# Autodesk Inventor assembly: NewChassis
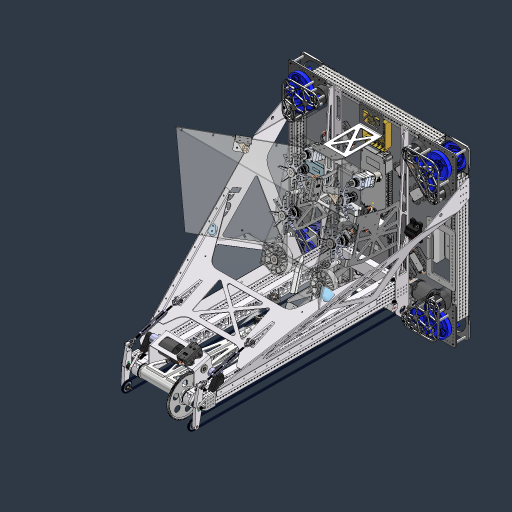
[picture p0: Inventor's stored thumbnail of the model, 512x512]
Saved by Autodesk Inventor 2024.3 (Build 283343000, 343)
## iProperties
ILogicPurgeVersion: 0.0.0.0
OnSaveVersion: 3.5.0.0
OnSaveAssembly: COREAutomationManager
Created: 2025-01-13
Part Number: NewChassis
Document SubType Name: Assembly
Designer: Marcus Tannini
Mfg Approved By: John.Thibert
Mass: 34331.5 g
Surface Area: 95241.2 cm^2
Volume: 13545.5 cm^3
Density: 2.53453 g/cm^3
ModelCat: Uncategorized
CN_MASS: 68.7
Author: Marcus Tannini
## Documents named in this file (42)
- D:\Inventor Projects\Poseidon V2\#Poseidon 2025.iam
- D:\Inventor Projects\Poseidon V2\ASSY,MK4i,Swerve_Module_INV.iam
- D:\Inventor Projects\Poseidon V2\MAXTube-2x1-Holes.ipt
- D:\Inventor Projects\Poseidon V2\BellyPanTop.ipt
- D:\Inventor Projects\Poseidon V2\BellyPanBot.ipt
- D:\Inventor Projects\Poseidon V2\BATTERY,12V.ipt
- D:\Inventor Projects\Poseidon V2\CONTROLS,MAIN_BREAKER.ipt
- D:\Inventor Projects\Poseidon V2\CONTROLS,MOTOR,NEO,550.ipt
- D:\Inventor Projects\Poseidon V2\CONTROLS,PDH.ipt
- D:\Inventor Projects\Poseidon V2\CONTROLS,PH.ipt
- D:\Inventor Projects\Poseidon V2\CONTROLS,ROBO_RIO.ipt
- D:\Inventor Projects\Poseidon V2\CONTROLS,SPARK_MAX.ipt
- D:\Inventor Projects\Poseidon V2\CONTROLS,VRM.ipt
- D:\Inventor Projects\Poseidon V2\COVER,SPARKMAX.ipt
- D:\Inventor Projects\Poseidon V2\ModifiedCase(IncludesPatterning).iam
- D:\Inventor Projects\Poseidon V2\PLATE,MOUNT,BATTERY,TOP.ipt
- D:\Inventor Projects\Poseidon V2\PLATE,MOUNT,BATTERY,BOT.ipt
- D:\Inventor Projects\Poseidon V2\MOUNT,STRAP,BATTERY.ipt
- D:\Inventor Projects\Poseidon V2\SPACER,SPROCKET,IDLER,ELEVATOR.ipt
- D:\Inventor Projects\Poseidon V2\PLATE,SIDE,BRACE,RIGHT,ELEVATOR.ipt
- D:\Inventor Projects\Poseidon V2\PLATE,SIDE,BRACE,LEFT,ELEVATOR.ipt
- D:\Inventor Projects\Poseidon V2\PLATE,TURNBUCKLE,TENSIONER,CHAIN.ipt
- D:\Inventor Projects\Poseidon V2\PLATE,BRACE,HORISONTAL,TOP,ELEVATOR.ipt
- D:\Inventor Projects\Poseidon V2\TURNBUCKLE,0.25IN_CLEVIS.iam
- D:\Inventor Projects\Poseidon V2\STAGE1,ELEVATOR.iam
- D:\Inventor Projects\Poseidon V2\ASSY,MAIN,ELEVATOR.iam
- D:\Inventor Projects\Poseidon V2\ANGLE,MOUNT,ELEVATOR.ipt
- D:\Inventor Projects\Poseidon V2\ANGLE,MOUNT,ELEVATOR,MIRR.ipt
- D:\Inventor Projects\Poseidon V2\FABRIC,BUMPERS.ipt
- D:\Inventor Projects\Poseidon V2\9293K119_Constant-Force Spring.ipt
- D:\Inventor Projects\Poseidon V2\MOUNT,SPRING,ELEVATOR.ipt
- D:\Inventor Projects\Poseidon V2\MOUNT,SPRING,ELEVATOR,MIRR.ipt
- D:\Inventor Projects\Poseidon V2\SPACER,HEX,0.125IN.ipt
- D:\Inventor Projects\Poseidon V2\ARM.iam
- D:\Inventor Projects\Poseidon V2\DRIVETRAIN,ELEVATOR.iam
- D:\Inventor Projects\Poseidon V2\hopper_assy.iam
- D:\Inventor Projects\Poseidon V2\feeder_front_support.ipt
- D:\Inventor Projects\Poseidon V2\coral_end_stop.ipt
- D:\Inventor Projects\Poseidon V2\coral_end_stop_MIR.ipt
- D:\Inventor Projects\Poseidon V2\hopper_backboard.ipt
- D:\Inventor Projects\Poseidon V2\Part Studio 1 - Support 1.ipt
- D:\Inventor Projects\Poseidon V2\Part Studio 1 - Support 2.ipt
## Components (67 placed, 43 different names)
1. FABRIC,BUMPERS.ipt:1 — Flush:323, Mate:335, Mate:336
2. hopper_assy:1 [sub-assembly] — Mate:656, Mate:657, Mate:658, Mate:671, Mate:672, Mate:673, Mate:674, Mate:675, Mate:676
3. feeder_front_support:1 — Mate:659, Mate:660, Mate:661, Mate:662, Mate:663, Mate:664, Mate:665, Mate:666, Mate:667
4. coral_end_stop:1 — Mate:665, Mate:666, Mate:667
5. coral_end_stop_MIR:1 — Mate:662, Mate:663, Mate:664
6. hopper_backboard:1 — Mate:668, Mate:669, Mate:670
7. Part Studio 1 - Support 1:1 — Mate:674, Mate:675, Mate:676
8. Part Studio 1 - Support 2:1 — Mate:671, Mate:672, Mate:673
9. ARM:1 [sub-assembly] — GEARS,ARM, Angle:1
10. COVER,SPARKMAX:9
11. CONTROLS,SPARK_MAX:9 — Mate:655
12. BellyPanBot.ipt:1 — Mate:66, Mate:353, Mate:354
13. BellyPanTop.ipt:1 — Mate:62, Mate:63, Mate:65, Mate:70, Mate:71, Mate:82, Mate:84, Insert:7, Insert:8, Insert:9, Insert:10, Insert:11, Insert:12, Insert:13, Insert:14, Insert:15, Insert:16, Insert:17, Insert:18, Insert:19, Insert:20, Insert:21, Insert:22, Mate:111, Mate:113, Mate:114, Mate:116, Mate:117, Mate:118, Mate:119, Mate:121, Mate:122, Mate:123, Mate:124, Mate:125, Mate:126, Mate:127, Mate:130, Insert:23, Insert:24, Mate:308, Mate:320, Mate:349, Mate:350, Mate:659, Mate:660, Mate:661
14. MAXTube-2x1-Holes.ipt:1 — Mate:1, Mate:2, Mate:3, Mate:4, Mate:5, Mate:15, Mate:115, Mate:272
15. MAXTube-2x1-Holes.ipt:2 — Mate:6, Mate:7, Mate:8, Mate:9, Mate:10, Mate:11, Mate:62, Mate:309, Mate:310
16. MAXTube-2x1-Holes.ipt:3 — Mate:19, Mate:20, Mate:21, Mate:66, Mate:114, Mate:312, Mate:313, Mate:336
17. MAXTube-2x1-Holes.ipt:4 — Mate:12, Mate:13, Mate:14, Mate:16, Mate:17, Mate:18, Mate:29, Mate:63, Mate:271, Mate:353, Mate:354
18. MOUNT,STRAP,BATTERY.ipt:1 — Mate:357, Mate:358, Mate:359
19. PLATE,MOUNT,BATTERY,BOT.ipt:1 — Mate:320, Mate:321, Mate:351, Mate:352
20. PLATE,MOUNT,BATTERY,TOP.ipt:1 — Mate:127, Mate:349, Mate:350, Mate:351, Mate:352, Mate:356, Mate:357, Mate:358, Mate:359
21. BATTERY,12V.ipt:1 — Mate:321, Mate:356
22. CONTROLS,MAIN_BREAKER.ipt:1 — Mate:82, Mate:111, Mate:116
23. CONTROLS,MOTOR,NEO,550.ipt:1
24. CONTROLS,PDH.ipt:1 — Mate:113, Mate:117, Mate:118, Mate:119
25. CONTROLS,PH.ipt:1 — Insert:23, Insert:24
26. CONTROLS,ROBO_RIO.ipt:1 — Mate:124, Mate:125, Mate:126
27. CONTROLS,SPARK_MAX.ipt:1 — Mate:84, Mate:85, Mate:86, Mate:87
28. CONTROLS,VRM.ipt:1 — Mate:121, Mate:122, Mate:123
29. ModifiedCase(IncludesPatterning).iam:1 [sub-assembly] — Mate:130
30. ASSY,MAIN,ELEVATOR.iam:1 [sub-assembly] — Mate:161, Mate:162, Flush:19, Mate:297, STAGE1 UPPER LIMIT, STAGE1 MAX, Mate:311, Mate:314, Mate:315, Mate:363, Mate:362, Mate:366, Mate:367, Mate:368, Mate:369
31. DRIVETRAIN,ELEVATOR:1 [sub-assembly]
32. STAGE1,ELEVATOR.iam:1 [sub-assembly] — Flush:19, Mate:297, STAGE1 LOWER LIMIT, STAGE1 UPPER LIMIT, STAGE1 MIN, STAGE1 MAX, GEARS,ARM, Angle:1, Mate:655
33. TURNBUCKLE,0.25IN_CLEVIS.iam:1 [sub-assembly]
34. TURNBUCKLE,0.25IN_CLEVIS.iam:2 [sub-assembly] — Mate:625
35. 9293K119_Constant-Force Spring:1 — Mate:364, Mate:365
36. 9293K119_Constant-Force Spring:2 — Mate:370, Mate:371
37. ANGLE,MOUNT,ELEVATOR,MIRR.ipt:1 — Mate:308, Mate:309, Mate:310, Mate:311, Mate:312, Mate:313, Mate:314, Mate:315, Mate:656, Mate:657, Mate:658
38. ANGLE,MOUNT,ELEVATOR.ipt:1 — Mate:65, Mate:70, Mate:71, Mate:161, Mate:162, STAGE1 LOWER LIMIT, STAGE1 MIN
39. MOUNT,SPRING,ELEVATOR,MIRR:1 — Mate:367, Mate:368, Mate:369, Mate:370, Mate:371
40. MOUNT,SPRING,ELEVATOR:1 — Mate:363, Mate:362, Mate:364, Mate:365, Mate:366
41. PLATE,BRACE,HORISONTAL,TOP,ELEVATOR.ipt:1 — Mate:285, Mate:286, Mate:289, Mate:290, Mate:291, Mate:295, Mate:296, Mate:668, Mate:669, Mate:670
42. PLATE,SIDE,BRACE,LEFT,ELEVATOR.ipt:1 — Mate:271, Mate:289, Mate:290, Mate:291, Mate:335
43. PLATE,SIDE,BRACE,RIGHT,ELEVATOR.ipt:1 — Mate:272
44. PLATE,TURNBUCKLE,TENSIONER,CHAIN.ipt:1 — Mate:285, Mate:296
45. PLATE,TURNBUCKLE,TENSIONER,CHAIN.ipt:2 — Mate:286, Mate:295, Mate:625
46. SPACER,HEX,0.125IN:1
47. SPACER,SPROCKET,IDLER,ELEVATOR.ipt:1
48. SPACER,SPROCKET,IDLER,ELEVATOR.ipt:2
49. ASSY,MK4i,Swerve_Module_INV.iam:1 [sub-assembly] — Mate:1, Mate:2, Mate:15
50. ASSY,MK4i,Swerve_Module_INV.iam:2 [sub-assembly] — Mate:3, Mate:4, Mate:5, Mate:6, Mate:7, Mate:8
51. ASSY,MK4i,Swerve_Module_INV.iam:3 [sub-assembly] — Mate:9, Mate:10, Mate:11, Mate:12, Mate:13, Mate:14
52. ASSY,MK4i,Swerve_Module_INV.iam:4 [sub-assembly] — Mate:16, Mate:17, Mate:18, Mate:19, Mate:20, Mate:21, Mate:67
53. CONTROLS,SPARK_MAX.ipt:2
54. CONTROLS,SPARK_MAX.ipt:3
55. CONTROLS,SPARK_MAX.ipt:4
56. CONTROLS,SPARK_MAX.ipt:5
57. CONTROLS,SPARK_MAX.ipt:6
58. CONTROLS,SPARK_MAX.ipt:7
59. CONTROLS,SPARK_MAX.ipt:8
60. COVER,SPARKMAX.ipt:1 — Mate:85, Mate:86, Mate:87, Insert:7, Insert:8
61. COVER,SPARKMAX.ipt:2 — Insert:9, Insert:10
62. COVER,SPARKMAX.ipt:3 — Insert:11, Insert:12
63. COVER,SPARKMAX.ipt:4 — Insert:13, Insert:14
64. COVER,SPARKMAX.ipt:5 — Insert:17, Insert:18
65. COVER,SPARKMAX.ipt:6 — Insert:15, Insert:16
66. COVER,SPARKMAX.ipt:7 — Insert:21, Insert:22
67. COVER,SPARKMAX.ipt:8 — Insert:19, Insert:20
## Relationships (198: Mate 170, Insert 22, Flush 4, RelateRotation 1, Angle 1)
- Mate:1: MAXTube-2x1-Holes.ipt:1 ↔ ASSY,MK4i,Swerve_Module_INV.iam:1
- Mate:2: MAXTube-2x1-Holes.ipt:1 ↔ ASSY,MK4i,Swerve_Module_INV.iam:1
- Mate:3: MAXTube-2x1-Holes.ipt:1 ↔ ASSY,MK4i,Swerve_Module_INV.iam:2
- Mate:4: MAXTube-2x1-Holes.ipt:1 ↔ ASSY,MK4i,Swerve_Module_INV.iam:2
- Mate:5: MAXTube-2x1-Holes.ipt:1 ↔ ASSY,MK4i,Swerve_Module_INV.iam:2
- Mate:6: MAXTube-2x1-Holes.ipt:2 ↔ ASSY,MK4i,Swerve_Module_INV.iam:2
- Mate:7: MAXTube-2x1-Holes.ipt:2 ↔ ASSY,MK4i,Swerve_Module_INV.iam:2
- Mate:8: MAXTube-2x1-Holes.ipt:2 ↔ ASSY,MK4i,Swerve_Module_INV.iam:2
- Mate:9: MAXTube-2x1-Holes.ipt:2 ↔ ASSY,MK4i,Swerve_Module_INV.iam:3
- Mate:10: MAXTube-2x1-Holes.ipt:2 ↔ ASSY,MK4i,Swerve_Module_INV.iam:3
- Mate:11: MAXTube-2x1-Holes.ipt:2 ↔ ASSY,MK4i,Swerve_Module_INV.iam:3
- Mate:12: MAXTube-2x1-Holes.ipt:4 ↔ ASSY,MK4i,Swerve_Module_INV.iam:3
- Mate:13: MAXTube-2x1-Holes.ipt:4 ↔ ASSY,MK4i,Swerve_Module_INV.iam:3
- Mate:14: MAXTube-2x1-Holes.ipt:4 ↔ ASSY,MK4i,Swerve_Module_INV.iam:3
- Mate:15: MAXTube-2x1-Holes.ipt:1 ↔ ASSY,MK4i,Swerve_Module_INV.iam:1
- Mate:16: MAXTube-2x1-Holes.ipt:4 ↔ ASSY,MK4i,Swerve_Module_INV.iam:4
- Mate:17: MAXTube-2x1-Holes.ipt:4 ↔ ASSY,MK4i,Swerve_Module_INV.iam:4
- Mate:18: MAXTube-2x1-Holes.ipt:4 ↔ ASSY,MK4i,Swerve_Module_INV.iam:4
- Mate:19: MAXTube-2x1-Holes.ipt:3 ↔ ASSY,MK4i,Swerve_Module_INV.iam:4
- Mate:20: MAXTube-2x1-Holes.ipt:3 ↔ ASSY,MK4i,Swerve_Module_INV.iam:4
- Mate:21: MAXTube-2x1-Holes.ipt:3 ↔ ASSY,MK4i,Swerve_Module_INV.iam:4
- Mate:29 (-6.35 mm): MAXTube-2x1-Holes.ipt:4
- Mate:62: BellyPanTop.ipt:1 ↔ MAXTube-2x1-Holes.ipt:2
- Mate:63: BellyPanTop.ipt:1 ↔ MAXTube-2x1-Holes.ipt:4
- Mate:65: BellyPanTop.ipt:1 ↔ ANGLE,MOUNT,ELEVATOR.ipt:1
- Mate:66: BellyPanBot.ipt:1 ↔ MAXTube-2x1-Holes.ipt:3
- Mate:67 (35.56 mm): ASSY,MK4i,Swerve_Module_INV.iam:4
- Mate:70: BellyPanTop.ipt:1 ↔ ANGLE,MOUNT,ELEVATOR.ipt:1
- Mate:71: BellyPanTop.ipt:1 ↔ ANGLE,MOUNT,ELEVATOR.ipt:1
- Mate:321: PLATE,MOUNT,BATTERY,BOT.ipt:1 ↔ BATTERY,12V.ipt:1
- Mate:82: BellyPanTop.ipt:1 ↔ CONTROLS,MAIN_BREAKER.ipt:1
- Mate:84: BellyPanTop.ipt:1 ↔ CONTROLS,SPARK_MAX.ipt:1
- Mate:85: CONTROLS,SPARK_MAX.ipt:1 ↔ COVER,SPARKMAX.ipt:1
- Mate:86: CONTROLS,SPARK_MAX.ipt:1 ↔ COVER,SPARKMAX.ipt:1
- Mate:87: CONTROLS,SPARK_MAX.ipt:1 ↔ COVER,SPARKMAX.ipt:1
- Insert:7: BellyPanTop.ipt:1 ↔ COVER,SPARKMAX.ipt:1
- Insert:8: BellyPanTop.ipt:1 ↔ COVER,SPARKMAX.ipt:1
- [Mate]: CONTROLS,SPARK_MAX.ipt:2 ↔ COVER,SPARKMAX.ipt:2
- [Mate]: CONTROLS,SPARK_MAX.ipt:2 ↔ COVER,SPARKMAX.ipt:2
- [Mate]: CONTROLS,SPARK_MAX.ipt:2 ↔ COVER,SPARKMAX.ipt:2
- [Mate]: CONTROLS,SPARK_MAX.ipt:3 ↔ COVER,SPARKMAX.ipt:3
- [Mate]: CONTROLS,SPARK_MAX.ipt:3 ↔ COVER,SPARKMAX.ipt:3
- [Mate]: CONTROLS,SPARK_MAX.ipt:3 ↔ COVER,SPARKMAX.ipt:3
- [Mate]: CONTROLS,SPARK_MAX.ipt:4 ↔ COVER,SPARKMAX.ipt:4
- [Mate]: CONTROLS,SPARK_MAX.ipt:4 ↔ COVER,SPARKMAX.ipt:4
- [Mate]: CONTROLS,SPARK_MAX.ipt:4 ↔ COVER,SPARKMAX.ipt:4
- [Mate]: CONTROLS,SPARK_MAX.ipt:5 ↔ COVER,SPARKMAX.ipt:5
- [Mate]: CONTROLS,SPARK_MAX.ipt:5 ↔ COVER,SPARKMAX.ipt:5
- [Mate]: CONTROLS,SPARK_MAX.ipt:5 ↔ COVER,SPARKMAX.ipt:5
- [Mate]: CONTROLS,SPARK_MAX.ipt:6 ↔ COVER,SPARKMAX.ipt:6
- [Mate]: CONTROLS,SPARK_MAX.ipt:6 ↔ COVER,SPARKMAX.ipt:6
- [Mate]: CONTROLS,SPARK_MAX.ipt:6 ↔ COVER,SPARKMAX.ipt:6
- [Mate]: CONTROLS,SPARK_MAX.ipt:7 ↔ COVER,SPARKMAX.ipt:7
- [Mate]: CONTROLS,SPARK_MAX.ipt:7 ↔ COVER,SPARKMAX.ipt:7
- [Mate]: CONTROLS,SPARK_MAX.ipt:7 ↔ COVER,SPARKMAX.ipt:7
- [Mate]: CONTROLS,SPARK_MAX.ipt:8 ↔ COVER,SPARKMAX.ipt:8
- [Mate]: CONTROLS,SPARK_MAX.ipt:8 ↔ COVER,SPARKMAX.ipt:8
- [Mate]: CONTROLS,SPARK_MAX.ipt:8 ↔ COVER,SPARKMAX.ipt:8
- Insert:9: BellyPanTop.ipt:1 ↔ COVER,SPARKMAX.ipt:2
- Insert:10: BellyPanTop.ipt:1 ↔ COVER,SPARKMAX.ipt:2
- Insert:11: BellyPanTop.ipt:1 ↔ COVER,SPARKMAX.ipt:3
- Insert:12: BellyPanTop.ipt:1 ↔ COVER,SPARKMAX.ipt:3
- Insert:13: BellyPanTop.ipt:1 ↔ COVER,SPARKMAX.ipt:4
- Insert:14: BellyPanTop.ipt:1 ↔ COVER,SPARKMAX.ipt:4
- Insert:15: BellyPanTop.ipt:1 ↔ COVER,SPARKMAX.ipt:6
- Insert:16: BellyPanTop.ipt:1 ↔ COVER,SPARKMAX.ipt:6
- Insert:17: BellyPanTop.ipt:1 ↔ COVER,SPARKMAX.ipt:5
- Insert:18: BellyPanTop.ipt:1 ↔ COVER,SPARKMAX.ipt:5
- Insert:19: BellyPanTop.ipt:1 ↔ COVER,SPARKMAX.ipt:8
- Insert:20: BellyPanTop.ipt:1 ↔ COVER,SPARKMAX.ipt:8
- Insert:21: BellyPanTop.ipt:1 ↔ COVER,SPARKMAX.ipt:7
- Insert:22: BellyPanTop.ipt:1 ↔ COVER,SPARKMAX.ipt:7
- Mate:111: BellyPanTop.ipt:1 ↔ CONTROLS,MAIN_BREAKER.ipt:1
- Mate:113: BellyPanTop.ipt:1 ↔ CONTROLS,PDH.ipt:1
- Mate:114: BellyPanTop.ipt:1 ↔ MAXTube-2x1-Holes.ipt:3
- Mate:115 (-374.65 mm): MAXTube-2x1-Holes.ipt:1
- Mate:116 (0.254 mm): BellyPanTop.ipt:1 ↔ CONTROLS,MAIN_BREAKER.ipt:1
- Mate:117: BellyPanTop.ipt:1 ↔ CONTROLS,PDH.ipt:1
- Mate:118: BellyPanTop.ipt:1 ↔ CONTROLS,PDH.ipt:1
- Mate:119: BellyPanTop.ipt:1 ↔ CONTROLS,PDH.ipt:1
- Mate:121: BellyPanTop.ipt:1 ↔ CONTROLS,VRM.ipt:1
- Mate:122: BellyPanTop.ipt:1 ↔ CONTROLS,VRM.ipt:1
- Mate:123: BellyPanTop.ipt:1 ↔ CONTROLS,VRM.ipt:1
- Mate:124: BellyPanTop.ipt:1 ↔ CONTROLS,ROBO_RIO.ipt:1
- Mate:125: BellyPanTop.ipt:1 ↔ CONTROLS,ROBO_RIO.ipt:1
- Mate:126: BellyPanTop.ipt:1 ↔ CONTROLS,ROBO_RIO.ipt:1
- Mate:127: BellyPanTop.ipt:1 ↔ PLATE,MOUNT,BATTERY,TOP.ipt:1
- Mate:130: BellyPanTop.ipt:1 ↔ ModifiedCase(IncludesPatterning).iam:1
- Insert:23: BellyPanTop.ipt:1 ↔ CONTROLS,PH.ipt:1
- Insert:24: BellyPanTop.ipt:1 ↔ CONTROLS,PH.ipt:1
- Mate:161: ASSY,MAIN,ELEVATOR.iam:1 ↔ ANGLE,MOUNT,ELEVATOR.ipt:1
- Mate:162: ASSY,MAIN,ELEVATOR.iam:1 ↔ ANGLE,MOUNT,ELEVATOR.ipt:1
- [Mate]: ASSY,MAIN,ELEVATOR.iam:1 ↔ ANGLE,MOUNT,ELEVATOR.ipt:1
- [Insert]: ASSY,MAIN,ELEVATOR.iam:1 ↔ SPACER,SPROCKET,IDLER,ELEVATOR.ipt:1
- [Insert]: ASSY,MAIN,ELEVATOR.iam:1 ↔ SPACER,SPROCKET,IDLER,ELEVATOR.ipt:1
- [Flush]: ASSY,MAIN,ELEVATOR.iam:1 ↔ DRIVETRAIN,ELEVATOR:1
- [Insert]: ASSY,MAIN,ELEVATOR.iam:1 ↔ SPACER,SPROCKET,IDLER,ELEVATOR.ipt:2
- [Insert]: ASSY,MAIN,ELEVATOR.iam:1 ↔ SPACER,SPROCKET,IDLER,ELEVATOR.ipt:2
- [Mate]: BellyPanTop.ipt:1 ↔ DRIVETRAIN,ELEVATOR:1
- [Mate]: DRIVETRAIN,ELEVATOR:1 ↔ ANGLE,MOUNT,ELEVATOR.ipt:1
- [Flush]: ASSY,MAIN,ELEVATOR.iam:1 ↔ DRIVETRAIN,ELEVATOR:1
- [Mate]: ASSY,MAIN,ELEVATOR.iam:1 ↔ PLATE,SIDE,BRACE,LEFT,ELEVATOR.ipt:1
- [Mate]: ASSY,MAIN,ELEVATOR.iam:1 ↔ PLATE,SIDE,BRACE,LEFT,ELEVATOR.ipt:1
- [Mate]: ASSY,MAIN,ELEVATOR.iam:1 ↔ DRIVETRAIN,ELEVATOR:1
- [Mate]: ASSY,MAIN,ELEVATOR.iam:1 ↔ PLATE,SIDE,BRACE,LEFT,ELEVATOR.ipt:1
- [Mate]: ASSY,MAIN,ELEVATOR.iam:1 ↔ PLATE,SIDE,BRACE,RIGHT,ELEVATOR.ipt:1
- [Mate]: ASSY,MAIN,ELEVATOR.iam:1 ↔ PLATE,SIDE,BRACE,RIGHT,ELEVATOR.ipt:1
- [Mate]: ASSY,MAIN,ELEVATOR.iam:1 ↔ PLATE,SIDE,BRACE,RIGHT,ELEVATOR.ipt:1
- Mate:271: MAXTube-2x1-Holes.ipt:4 ↔ PLATE,SIDE,BRACE,LEFT,ELEVATOR.ipt:1
- Mate:272: MAXTube-2x1-Holes.ipt:1 ↔ PLATE,SIDE,BRACE,RIGHT,ELEVATOR.ipt:1
- [Mate]: ASSY,MAIN,ELEVATOR.iam:1 ↔ TURNBUCKLE,0.25IN_CLEVIS.iam:1
- [Mate]: ASSY,MAIN,ELEVATOR.iam:1 ↔ TURNBUCKLE,0.25IN_CLEVIS.iam:1
- [Mate]: ASSY,MAIN,ELEVATOR.iam:1 ↔ TURNBUCKLE,0.25IN_CLEVIS.iam:2
- [Mate]: ASSY,MAIN,ELEVATOR.iam:1 ↔ TURNBUCKLE,0.25IN_CLEVIS.iam:2
- Mate:285: PLATE,BRACE,HORISONTAL,TOP,ELEVATOR.ipt:1 ↔ PLATE,TURNBUCKLE,TENSIONER,CHAIN.ipt:1
- Mate:286: PLATE,BRACE,HORISONTAL,TOP,ELEVATOR.ipt:1 ↔ PLATE,TURNBUCKLE,TENSIONER,CHAIN.ipt:2
- Mate:289: PLATE,BRACE,HORISONTAL,TOP,ELEVATOR.ipt:1 ↔ PLATE,SIDE,BRACE,LEFT,ELEVATOR.ipt:1
- Mate:290: PLATE,BRACE,HORISONTAL,TOP,ELEVATOR.ipt:1 ↔ PLATE,SIDE,BRACE,LEFT,ELEVATOR.ipt:1
- Mate:291: PLATE,BRACE,HORISONTAL,TOP,ELEVATOR.ipt:1 ↔ PLATE,SIDE,BRACE,LEFT,ELEVATOR.ipt:1
- [Mate]: ASSY,MAIN,ELEVATOR.iam:1 ↔ DRIVETRAIN,ELEVATOR:1
- Mate:295: PLATE,BRACE,HORISONTAL,TOP,ELEVATOR.ipt:1 ↔ PLATE,TURNBUCKLE,TENSIONER,CHAIN.ipt:2
- Mate:296: PLATE,BRACE,HORISONTAL,TOP,ELEVATOR.ipt:1 ↔ PLATE,TURNBUCKLE,TENSIONER,CHAIN.ipt:1
- Flush:19: ASSY,MAIN,ELEVATOR.iam:1 ↔ STAGE1,ELEVATOR.iam:1
- Mate:297: ASSY,MAIN,ELEVATOR.iam:1 ↔ STAGE1,ELEVATOR.iam:1
- STAGE1 LOWER LIMIT [Mate]: STAGE1,ELEVATOR.iam:1 ↔ ANGLE,MOUNT,ELEVATOR.ipt:1
- STAGE1 UPPER LIMIT [Mate]: ASSY,MAIN,ELEVATOR.iam:1 ↔ STAGE1,ELEVATOR.iam:1
- STAGE1 MIN [Mate]: STAGE1,ELEVATOR.iam:1 ↔ ANGLE,MOUNT,ELEVATOR.ipt:1
- STAGE1 MAX [Mate] (3.175 mm): ASSY,MAIN,ELEVATOR.iam:1 ↔ STAGE1,ELEVATOR.iam:1
- Mate:308: BellyPanTop.ipt:1 ↔ ANGLE,MOUNT,ELEVATOR,MIRR.ipt:1
- Mate:309: MAXTube-2x1-Holes.ipt:2 ↔ ANGLE,MOUNT,ELEVATOR,MIRR.ipt:1
- Mate:310: MAXTube-2x1-Holes.ipt:2 ↔ ANGLE,MOUNT,ELEVATOR,MIRR.ipt:1
- Mate:311: ASSY,MAIN,ELEVATOR.iam:1 ↔ ANGLE,MOUNT,ELEVATOR,MIRR.ipt:1
- Mate:312: MAXTube-2x1-Holes.ipt:3 ↔ ANGLE,MOUNT,ELEVATOR,MIRR.ipt:1
- Mate:313: MAXTube-2x1-Holes.ipt:3 ↔ ANGLE,MOUNT,ELEVATOR,MIRR.ipt:1
- Mate:314: ASSY,MAIN,ELEVATOR.iam:1 ↔ ANGLE,MOUNT,ELEVATOR,MIRR.ipt:1
- Mate:315: ASSY,MAIN,ELEVATOR.iam:1 ↔ ANGLE,MOUNT,ELEVATOR,MIRR.ipt:1
- Mate:320: BellyPanTop.ipt:1 ↔ PLATE,MOUNT,BATTERY,BOT.ipt:1
- Flush:323 (146.05 mm): FABRIC,BUMPERS.ipt:1
- Mate:335 (3.175 mm): FABRIC,BUMPERS.ipt:1 ↔ PLATE,SIDE,BRACE,LEFT,ELEVATOR.ipt:1
- Mate:336 (6.35 mm): FABRIC,BUMPERS.ipt:1 ↔ MAXTube-2x1-Holes.ipt:3
- Mate:349: BellyPanTop.ipt:1 ↔ PLATE,MOUNT,BATTERY,TOP.ipt:1
- Mate:350: BellyPanTop.ipt:1 ↔ PLATE,MOUNT,BATTERY,TOP.ipt:1
- Mate:351: PLATE,MOUNT,BATTERY,BOT.ipt:1 ↔ PLATE,MOUNT,BATTERY,TOP.ipt:1
- Mate:352: PLATE,MOUNT,BATTERY,BOT.ipt:1 ↔ PLATE,MOUNT,BATTERY,TOP.ipt:1
- Mate:353: BellyPanBot.ipt:1 ↔ MAXTube-2x1-Holes.ipt:4
- Mate:354: BellyPanBot.ipt:1 ↔ MAXTube-2x1-Holes.ipt:4
- Mate:356 (19.05 mm): PLATE,MOUNT,BATTERY,TOP.ipt:1 ↔ BATTERY,12V.ipt:1
- Mate:357: MOUNT,STRAP,BATTERY.ipt:1 ↔ PLATE,MOUNT,BATTERY,TOP.ipt:1
- Mate:358: MOUNT,STRAP,BATTERY.ipt:1 ↔ PLATE,MOUNT,BATTERY,TOP.ipt:1
- Mate:359: MOUNT,STRAP,BATTERY.ipt:1 ↔ PLATE,MOUNT,BATTERY,TOP.ipt:1
- Mate:363: ASSY,MAIN,ELEVATOR.iam:1 ↔ MOUNT,SPRING,ELEVATOR:1
- Mate:362: ASSY,MAIN,ELEVATOR.iam:1 ↔ MOUNT,SPRING,ELEVATOR:1
- Mate:364: 9293K119_Constant-Force Spring:1 ↔ MOUNT,SPRING,ELEVATOR:1
- Mate:365 (1.5875 mm): 9293K119_Constant-Force Spring:1 ↔ MOUNT,SPRING,ELEVATOR:1
- Mate:366: ASSY,MAIN,ELEVATOR.iam:1 ↔ MOUNT,SPRING,ELEVATOR:1
- Mate:367: ASSY,MAIN,ELEVATOR.iam:1 ↔ MOUNT,SPRING,ELEVATOR,MIRR:1
- Mate:368: ASSY,MAIN,ELEVATOR.iam:1 ↔ MOUNT,SPRING,ELEVATOR,MIRR:1
- Mate:369: ASSY,MAIN,ELEVATOR.iam:1 ↔ MOUNT,SPRING,ELEVATOR,MIRR:1
- Mate:370: 9293K119_Constant-Force Spring:2 ↔ MOUNT,SPRING,ELEVATOR,MIRR:1
- Mate:371 (1.5875 mm): 9293K119_Constant-Force Spring:2 ↔ MOUNT,SPRING,ELEVATOR,MIRR:1
- [Mate] (0.254 mm): ASSY,MAIN,ELEVATOR.iam:1 ↔ DRIVETRAIN,ELEVATOR:1
- [Mate]: ASSY,MAIN,ELEVATOR.iam:1 ↔ DRIVETRAIN,ELEVATOR:1
- [Mate]: DRIVETRAIN,ELEVATOR:1 ↔ SPACER,HEX,0.125IN:1
- [Mate]: DRIVETRAIN,ELEVATOR:1 ↔ SPACER,HEX,0.125IN:1
- [Mate]: ARM:1 ↔ STAGE1,ELEVATOR.iam:1
- [Mate]: ARM:1 ↔ STAGE1,ELEVATOR.iam:1
- [Mate]: MAXTube-2x1-Holes.ipt:2 ↔ DRIVETRAIN,ELEVATOR:1
- [Mate]: MAXTube-2x1-Holes.ipt:2 ↔ DRIVETRAIN,ELEVATOR:1
- Mate:625 (1.524 mm): TURNBUCKLE,0.25IN_CLEVIS.iam:2 ↔ PLATE,TURNBUCKLE,TENSIONER,CHAIN.ipt:2
- [Mate]: ARM:1 ↔ STAGE1,ELEVATOR.iam:1
- [Mate]: ARM:1 ↔ STAGE1,ELEVATOR.iam:1
- GEARS,ARM [RelateRotation] (4.5 ul): ARM:1 ↔ STAGE1,ELEVATOR.iam:1
- Angle:1 (0 deg): ARM:1 ↔ STAGE1,ELEVATOR.iam:1
- [Mate]: COVER,SPARKMAX:9 ↔ CONTROLS,SPARK_MAX:9
- [Mate]: COVER,SPARKMAX:9 ↔ CONTROLS,SPARK_MAX:9
- [Mate]: COVER,SPARKMAX:9 ↔ CONTROLS,SPARK_MAX:9
- Mate:655: CONTROLS,SPARK_MAX:9 ↔ STAGE1,ELEVATOR.iam:1
- Mate:656: hopper_assy:1 ↔ ANGLE,MOUNT,ELEVATOR,MIRR.ipt:1
- Mate:657: hopper_assy:1 ↔ ANGLE,MOUNT,ELEVATOR,MIRR.ipt:1
- Mate:658: hopper_assy:1 ↔ ANGLE,MOUNT,ELEVATOR,MIRR.ipt:1
- Mate:659: feeder_front_support:1 ↔ BellyPanTop.ipt:1
- Mate:660: feeder_front_support:1 ↔ BellyPanTop.ipt:1
- Mate:661: feeder_front_support:1 ↔ BellyPanTop.ipt:1
- Mate:662: feeder_front_support:1 ↔ coral_end_stop_MIR:1
- Mate:663: feeder_front_support:1 ↔ coral_end_stop_MIR:1
- Mate:664: feeder_front_support:1 ↔ coral_end_stop_MIR:1
- Mate:665: feeder_front_support:1 ↔ coral_end_stop:1
- Mate:666: feeder_front_support:1 ↔ coral_end_stop:1
- Mate:667: feeder_front_support:1 ↔ coral_end_stop:1
- Mate:668: hopper_backboard:1 ↔ PLATE,BRACE,HORISONTAL,TOP,ELEVATOR.ipt:1
- Mate:669: hopper_backboard:1 ↔ PLATE,BRACE,HORISONTAL,TOP,ELEVATOR.ipt:1
- Mate:670: hopper_backboard:1 ↔ PLATE,BRACE,HORISONTAL,TOP,ELEVATOR.ipt:1
- Mate:671: hopper_assy:1 ↔ Part Studio 1 - Support 2:1
- Mate:672: hopper_assy:1 ↔ Part Studio 1 - Support 2:1
- Mate:673: hopper_assy:1 ↔ Part Studio 1 - Support 2:1
- Mate:674: hopper_assy:1 ↔ Part Studio 1 - Support 1:1
- Mate:675: hopper_assy:1 ↔ Part Studio 1 - Support 1:1
- Mate:676: hopper_assy:1 ↔ Part Studio 1 - Support 1:1
## Named parameters: d160_d155 = 0 mm, d161_d156 = 0 mm, d162_d157 = 0 mm, d163_d155 = 0 mm, d164_d156 = 0 mm, d165_d157 = 0 mm, d166_d155 = 0 mm, d167_d156 = 0 mm, d168_d157 = 0 mm, d169_d155 = 0 mm, d170_d156 = 0 mm, d171_d157 = 0 mm, d172_d155 = 0 mm, d173_d156 = 0 mm, d174_d157 = 0 mm, d175_d155 = 0 mm, d176_d156 = 0 mm, d177_d157 = 0 mm, d178_d155 = 0 mm, d179_d156 = 0 mm, d180_d157 = 0 mm, d518_d513 = 0 mm, d1392_d178_d155 = 0 mm, d1393_d179_d156 = 0 mm, d1394_d180_d157 = 0 mm
